# Autodesk Inventor assembly: WheelAssembly
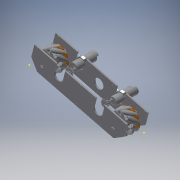
[picture p0: Inventor's stored thumbnail of the model, 180x180]
Saved by Autodesk Inventor 2017 (Build 210142000, 142)
## iProperties
Created: 2016-09-10
Part Number: WheelAssembly
Document SubType Name: Assembly
Designer: RoboticsUser
Author: RoboticsUser
## Documents named in this file (10)
- C:\Robotics\CAD\2016-17_CAD\WheelAssemble2.0.iam
- C:\Robotics\CAD\COTSParts\Actobotics\545 parts\545556.ipt
- C:\Robotics\CAD\COTSParts\Actobotics\615 parts\615102.ipt
- C:\Robotics\CAD\COTSParts\Actobotics\634 parts\634080.ipt
- C:\Robotics\CAD\COTSParts\Motors\Andymark 2964  NeveRest 40 Motor.ipt
- C:\Robotics\CAD\COTSParts\Tetrix\tetrix-motor-mounts-1.snapshot.1\Tetrex 2pc motor mount.ipt
- C:\Robotics\CAD\2016-17_CAD\DriveTrainPlateInside1.iam
- C:\Robotics\CAD\COTSParts\Actobotics\545 parts\545456.ipt
- C:\Robotics\CAD\2016-17_CAD\DriveTrainPlateOutside2.iam
- C:\Robotics\CAD\COTSParts\Wheels\AndyMark Mecanum Wheels\100mm Aluminum Mecanum wheels.ipt
## Components (22 placed, 9 different names)
1. 545556:2 — Mate:10, Mate:11, Mate:13
2. 615102:4 — Mate:18, Mate:19, Flush:2
3. 634080:2 — Insert:70, Mate:10, Mate:12, Mate:21, Insert:91, Mate:23
4. 545556:6 — Insert:82, Insert:83
5. 615102:5 — Insert:86, Mate:2
6. 634080:3 — Insert:66, Insert:82, Insert:90
7. Andymark 2964  NeveRest 40 Motor:2 — Mate:1, Mate:3
8. 545556:8 — Mate:1, Mate:2, Mate:4
9. 545556:9 — Mate:7, Mate:18
10. Andymark 2964  NeveRest 40 Motor:3 — Mate:7, Mate:19
11. Tetrex 2pc motor mount:1 — Insert:92
12. Tetrex 2pc motor mount:2 — Insert:93
13. DriveTrainPlateInside1:1 [sub-assembly] — Insert:66, Insert:70, Mate:11, Mate:22, Insert:92, Insert:93
14. 545556:10 — Insert:87
15. 545456:1 — Mate:12, Mate:13, Insert:89
16. 545456:3 — Insert:83, Insert:88
17. 545556:11 — Insert:86
18. DriveTrainPlateOutside2:1 [sub-assembly] — Mate:22, Insert:90, Insert:91, Mate:23
19. 615102:6 — Mate:3, Mate:4
20. 615102:7 — Mate:21, Insert:87, Flush:2
21. 100mm Aluminum Mecanum wheels:1 — Insert:88
22. 100mm Aluminum Mecanum wheels:2 — Insert:89
## Relationships (27: Mate 14, Insert 12, Flush 1)
- Insert:66 (-6.35 mm): 634080:3 ↔ DriveTrainPlateInside1:1
- Insert:70 (-6.35 mm): 634080:2 ↔ DriveTrainPlateInside1:1
- Insert:82 (12.7 mm): 545556:6 ↔ 634080:3
- Insert:83: 545556:6 ↔ 545456:3
- Insert:86: 615102:5 ↔ 545556:11
- Mate:1: Andymark 2964  NeveRest 40 Motor:2 ↔ 545556:8
- Mate:2: 615102:5 ↔ 545556:8
- Mate:3: Andymark 2964  NeveRest 40 Motor:2 ↔ 615102:6
- Mate:4: 545556:8 ↔ 615102:6
- Mate:7: 545556:9 ↔ Andymark 2964  NeveRest 40 Motor:3
- Mate:10: 545556:2 ↔ 634080:2
- Mate:11: 545556:2 ↔ DriveTrainPlateInside1:1
- Mate:12: 634080:2 ↔ 545456:1
- Mate:13: 545556:2 ↔ 545456:1
- Mate:18: 615102:4 ↔ 545556:9
- Mate:19: 615102:4 ↔ Andymark 2964  NeveRest 40 Motor:3
- Mate:21: 634080:2 ↔ 615102:7
- Insert:87: 545556:10 ↔ 615102:7
- Flush:2: 615102:4 ↔ 615102:7
- Insert:88: 545456:3 ↔ 100mm Aluminum Mecanum wheels:1
- Insert:89: 545456:1 ↔ 100mm Aluminum Mecanum wheels:2
- Mate:22 (91.2622 mm): DriveTrainPlateInside1:1 ↔ DriveTrainPlateOutside2:1
- Insert:90: 634080:3 ↔ DriveTrainPlateOutside2:1
- Insert:91: 634080:2 ↔ DriveTrainPlateOutside2:1
- Mate:23: 634080:2 ↔ DriveTrainPlateOutside2:1
- Insert:92: Tetrex 2pc motor mount:1 ↔ DriveTrainPlateInside1:1
- Insert:93: Tetrex 2pc motor mount:2 ↔ DriveTrainPlateInside1:1
